# Autodesk Inventor assembly: TwoWheelBlock
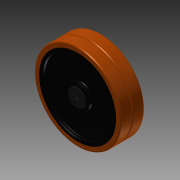
[picture p0: Inventor's stored thumbnail of the model, 180x180]
Saved by Autodesk Inventor 2014 SP1 (Build 180222100, 222)
## iProperties
Created: 2015-04-11
Part Number: TwoWheelBlock
Document SubType Name: Assembly
Designer: david
Author: david
## Documents named in this file (3)
- C:\Users\asus\Documents\Autodesk\Projects\AUSBEEDone\Components\BaneBots\TwoWheelBlock.iam
- C:\Users\asus\Documents\Autodesk\Projects\AUSBEEDone\Components\BaneBots\Hub_Hex_4mmBore_2Wide.ipt
- C:\Users\asus\Documents\Autodesk\Projects\AUSBEEDone\Components\BaneBots\Wheel_73mm-10mm-HexMount_40A.ipt
## Components (3 placed, 2 different names)
1. Hub_Hex_4mmBore_2Wide:1 — Mate:1, Mate:2, Mate:3, Mate:4, Mate:5
2. Wheel_73mm-10mm-HexMount_40A:1 — Mate:1, Mate:4, Mate:5, Mate:6
3. Wheel_73mm-10mm-HexMount_40A:2 — Mate:2, Mate:3, Mate:6
## Relationships (6: Mate 6)
- Mate:1: Hub_Hex_4mmBore_2Wide:1 ↔ Wheel_73mm-10mm-HexMount_40A:1
- Mate:2: Hub_Hex_4mmBore_2Wide:1 ↔ Wheel_73mm-10mm-HexMount_40A:2
- Mate:3: Hub_Hex_4mmBore_2Wide:1 ↔ Wheel_73mm-10mm-HexMount_40A:2
- Mate:4: Hub_Hex_4mmBore_2Wide:1 ↔ Wheel_73mm-10mm-HexMount_40A:1
- Mate:5: Hub_Hex_4mmBore_2Wide:1 ↔ Wheel_73mm-10mm-HexMount_40A:1
- Mate:6: Wheel_73mm-10mm-HexMount_40A:1 ↔ Wheel_73mm-10mm-HexMount_40A:2
